# Autodesk Inventor assembly: Assembly1
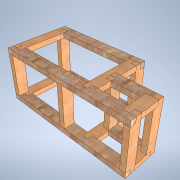
[picture p0: Inventor's stored thumbnail of the model, 180x180]
Saved by Autodesk Inventor 2022 (Build 260153000, 153)
## iProperties
Created: 2021-12-11
Part Number: Assembly1
Document SubType Name: Assembly
Designer: dangl
Author: dangl
## Documents named in this file (7)
- C:\Users\dangl\Documents\WoodWork\WorkBench\Assembly1.iam
- C:\Users\dangl\Documents\WoodWork\WorkBench\beam1.ipt
- C:\Users\dangl\Documents\WoodWork\WorkBench\beam2.ipt
- C:\Users\dangl\Documents\WoodWork\WorkBench\beam3.ipt
- C:\Users\dangl\Documents\WoodWork\WorkBench\beam4.ipt
- C:\Users\dangl\Documents\WoodWork\WorkBench\beam5.ipt
- C:\Users\dangl\Documents\WoodWork\WorkBench\beam6.ipt
## Components (19 placed, 6 different names)
1. beam1:1 — Mate:4, Mate:5, Mate:6, Flush:1, Flush:9, Mate:11, Mate:12, Flush:12, Mate:13, Flush:19
2. beam1:2 — Mate:1, Mate:2, Mate:3, Flush:2, Flush:3, Flush:4, Flush:5, Flush:6, Flush:8, Mate:8, Flush:11, Mate:9, Mate:10, Flush:15
3. beam2:1 — Mate:1, Mate:2, Mate:3, Mate:4, Mate:5, Mate:6
4. beam2:2 — Flush:1, Flush:2, Flush:3, Flush:13, Flush:14, Mate:14
5. beam2:3 — Flush:4, Flush:5, Flush:6, Flush:7, Mate:7, Flush:10
6. beam2:4 — Flush:9, Mate:7, Flush:10, Mate:22, Flush:30
7. beam2:5 — Flush:7, Flush:8, Mate:8, Flush:31
8. beam3:1 — Flush:11, Mate:9, Mate:10, Flush:22, Mate:18, Mate:19
9. beam3:2 — Mate:11, Mate:12, Mate:17, Flush:19, Flush:23, Mate:21, Flush:25, Mate:23
10. beam4:1 — Flush:12, Mate:13, Flush:13, Flush:16, Mate:15, Flush:17, Flush:18
11. beam4:2 — Flush:14, Flush:15, Mate:14
12. beam2:6 — Flush:16, Mate:15, Flush:17, Flush:20, Flush:21
13. beam5:1 — Flush:18, Mate:17, Flush:20, Flush:24
14. beam5:2 — Flush:21, Flush:22, Mate:18
15. beam2:7 — Flush:23, Flush:24, Mate:19
16. beam6:1 — Mate:21, Flush:25, Mate:22, Flush:26, Flush:27, Flush:28, Flush:29
17. beam2:8 — Mate:23, Flush:26, Flush:27
18. beam2:9 — Flush:28, Flush:29, Flush:30, Flush:32, Flush:33
19. beam6:2 — Flush:31, Flush:32, Flush:33
## Relationships (54: Flush 33, Mate 21)
- Mate:1: beam1:2 ↔ beam2:1
- Mate:2: beam1:2 ↔ beam2:1
- Mate:3: beam1:2 ↔ beam2:1
- Mate:4: beam1:1 ↔ beam2:1
- Mate:5: beam1:1 ↔ beam2:1
- Mate:6: beam1:1 ↔ beam2:1
- Flush:1: beam1:1 ↔ beam2:2
- Flush:2: beam1:2 ↔ beam2:2
- Flush:3: beam1:2 ↔ beam2:2
- Flush:4: beam1:2 ↔ beam2:3
- Flush:5: beam1:2 ↔ beam2:3
- Flush:6: beam1:2 ↔ beam2:3
- Flush:7: beam2:3 ↔ beam2:5
- Flush:8: beam1:2 ↔ beam2:5
- Flush:9: beam1:1 ↔ beam2:4
- Mate:7: beam2:3 ↔ beam2:4
- Flush:10: beam2:3 ↔ beam2:4
- Mate:8: beam1:2 ↔ beam2:5
- Flush:11: beam1:2 ↔ beam3:1
- Mate:9: beam1:2 ↔ beam3:1
- Mate:10: beam1:2 ↔ beam3:1
- Mate:11: beam1:1 ↔ beam3:2
- Mate:12: beam1:1 ↔ beam3:2
- Flush:12: beam1:1 ↔ beam4:1
- Mate:13: beam1:1 ↔ beam4:1
- Flush:13: beam2:2 ↔ beam4:1
- Flush:14: beam2:2 ↔ beam4:2
- Flush:15: beam1:2 ↔ beam4:2
- Mate:14: beam2:2 ↔ beam4:2
- Flush:16: beam4:1 ↔ beam2:6
- Mate:15: beam4:1 ↔ beam2:6
- Flush:17: beam4:1 ↔ beam2:6
- Flush:18: beam4:1 ↔ beam5:1
- Mate:17: beam3:2 ↔ beam5:1
- Flush:19: beam1:1 ↔ beam3:2
- Flush:20: beam2:6 ↔ beam5:1
- Flush:21: beam2:6 ↔ beam5:2
- Flush:22: beam3:1 ↔ beam5:2
- Mate:18: beam3:1 ↔ beam5:2
- Flush:23: beam3:2 ↔ beam2:7
- Flush:24: beam5:1 ↔ beam2:7
- Mate:19: beam3:1 ↔ beam2:7
- Mate:21: beam3:2 ↔ beam6:1
- Flush:25: beam3:2 ↔ beam6:1
- Mate:22: beam2:4 ↔ beam6:1
- Mate:23: beam3:2 ↔ beam2:8
- Flush:26: beam6:1 ↔ beam2:8
- Flush:27: beam6:1 ↔ beam2:8
- Flush:28: beam6:1 ↔ beam2:9
- Flush:29: beam6:1 ↔ beam2:9
- Flush:30: beam2:4 ↔ beam2:9
- Flush:31: beam2:5 ↔ beam6:2
- Flush:32: beam2:9 ↔ beam6:2
- Flush:33: beam2:9 ↔ beam6:2
